# Autodesk Inventor assembly: Idler pulley kit
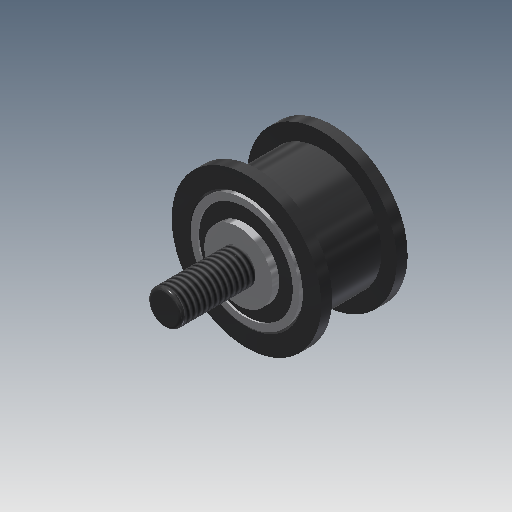
[picture p0: Inventor's stored thumbnail of the model, 512x512]
Saved by Autodesk Inventor 2020.3 (Build 243373000, 373)
## iProperties
Created: 2016-04-12
Part Number: Idler pulley kit
Document SubType Name: Assembly
Designer: Ben
Author: Ben
## Documents named in this file (6)
- F:\UQ Engineering\2021 ~ 5th Year\Semester 2\METR4911-THESIS\FarmBot CAD\FarmBotV1\VSlotHardware\Idler pulley kit.iam
- F:\UQ Engineering\2021 ~ 5th Year\Semester 2\METR4911-THESIS\FarmBot CAD\FarmBotV1\VSlotHardware\M5x25 low profile screw.ipt
- F:\UQ Engineering\2021 ~ 5th Year\Semester 2\METR4911-THESIS\FarmBot CAD\FarmBotV1\VSlotHardware\Ball Bearing 625 2RS 5x16x5.ipt
- F:\UQ Engineering\2021 ~ 5th Year\Semester 2\METR4911-THESIS\FarmBot CAD\FarmBotV1\VSlotHardware\1mm 5mm shim.ipt
- F:\UQ Engineering\2021 ~ 5th Year\Semester 2\METR4911-THESIS\FarmBot CAD\FarmBotV1\VSlotHardware\Nylon Spacer 1_8th.ipt
- F:\UQ Engineering\2021 ~ 5th Year\Semester 2\METR4911-THESIS\FarmBot CAD\FarmBotV1\VSlotHardware\idler pulley.ipt
## Components (6 placed, 5 different names)
1. M5x25 low profile screw:1 — Mate:1, Mate:2, Flush:1, Mate:3, Mate:4, Mate:5, Mate:6, Mate:7
2. Ball Bearing 625 2RS 5x16x5:1 — Mate:3, Mate:10, Mate:12, Mate:13
3. Ball Bearing 625 2RS 5x16x5:2 — Mate:4, Mate:5, Mate:8, Mate:11
4. 1mm 5mm shim:1 — Mate:6, Mate:13
5. Nylon Spacer 1_8th:1 — Mate:7, Mate:8
6. idler pulley:1 — Mate:10, Mate:11, Mate:12
## Relationships (13: Mate 12, Flush 1)
- Mate:1: M5x25 low profile screw:1
- Mate:2: M5x25 low profile screw:1
- Flush:1: M5x25 low profile screw:1
- Mate:3: M5x25 low profile screw:1 ↔ Ball Bearing 625 2RS 5x16x5:1
- Mate:4: M5x25 low profile screw:1 ↔ Ball Bearing 625 2RS 5x16x5:2
- Mate:5: M5x25 low profile screw:1 ↔ Ball Bearing 625 2RS 5x16x5:2
- Mate:6: M5x25 low profile screw:1 ↔ 1mm 5mm shim:1
- Mate:7: M5x25 low profile screw:1 ↔ Nylon Spacer 1_8th:1
- Mate:8: Ball Bearing 625 2RS 5x16x5:2 ↔ Nylon Spacer 1_8th:1
- Mate:10: Ball Bearing 625 2RS 5x16x5:1 ↔ idler pulley:1
- Mate:11: Ball Bearing 625 2RS 5x16x5:2 ↔ idler pulley:1
- Mate:12: Ball Bearing 625 2RS 5x16x5:1 ↔ idler pulley:1
- Mate:13: Ball Bearing 625 2RS 5x16x5:1 ↔ 1mm 5mm shim:1
